# Autodesk Inventor assembly: søjle+vange
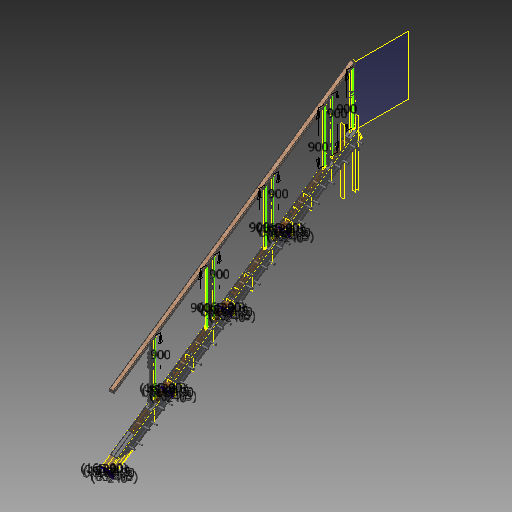
[picture p0: Inventor's stored thumbnail of the model, 512x512]
Saved by Autodesk Inventor 2018 (Build 220112000, 112)
## iProperties
Created: 2019-09-25
Part Number: søjle+vange
Document SubType Name: Assembly
Designer: Kristoffer Ek
Mass: 165952 g
Surface Area: 103178 cm^2
Volume: 42097.6 cm^3
Density: 3.94208 g/cm^3
Description: Beplantet bæredygtig trappe
Engineer: Kristoffer Ek
Authority: Loppen
Author: Kristoffer Ek
Title: Beplantet bæredygtig trappe
## Documents named in this file (35)
- Z:\trappe\søjle+vange.iam
- Z:\trappe\modul top.iam
- Z:\trappe\søjle\stilladssøjle.iam
- Z:\trappe\modul.iam
- Z:\trappe\modul bund.iam
- Z:\trappe\håndfang\træhåndfang.ipt
- Z:\trappe\hegn\hegnspæl.iam
- Z:\trappe\hegn\hegnspæl omvendt.iam
- Z:\trappe\søjle+vange\Design Accelerator\Bolted Connection1.iam
- Z:\trappe\søjle+vange\Design Accelerator\Bolted Connection2.iam
- Z:\trappe\søjle+vange\Design Accelerator\Bolted Connection3.iam
- Z:\trappe\søjle+vange\Design Accelerator\Bolted Connection4.iam
- Z:\trappe\søjle+vange\Design Accelerator\Bolted Connection5.iam
- Z:\trappe\søjle+vange\Design Accelerator\Bolted Connection6.iam
- Z:\trappe\søjle+vange\Design Accelerator\Bolted Connection7.iam
- Z:\trappe\søjle+vange\Design Accelerator\Bolted Connection8.iam
- Z:\trappe\søjle+vange\Design Accelerator\Bolted Connection9.iam
- Z:\trappe\søjle+vange\Design Accelerator\Bolted Connection10.iam
- Z:\trappe\søjle+vange\Design Accelerator\Bolted Connection11.iam
- Z:\trappe\søjle+vange\Design Accelerator\Bolted Connection12.iam
- Z:\trappe\søjle+vange\Design Accelerator\Bolted Connection13.iam
- Z:\trappe\søjle+vange\Design Accelerator\Bolted Connection14.iam
- Z:\trappe\søjle+vange\Design Accelerator\Bolted Connection15.iam
- Z:\trappe\søjle+vange\Design Accelerator\Bolted Connection16.iam
- Z:\trappe\søjle+vange\Design Accelerator\Bolted Connection17.iam
- Z:\trappe\søjle+vange\Design Accelerator\Bolted Connection18.iam
- Z:\trappe\søjle+vange\Design Accelerator\Bolted Connection19.iam
- Z:\trappe\søjle+vange\Design Accelerator\Bolted Connection20.iam
- Z:\trappe\søjle+vange\Design Accelerator\Bolted Connection21.iam
- Z:\trappe\søjle+vange\Design Accelerator\Bolted Connection22.iam
- Z:\trappe\søjle+vange\Design Accelerator\Bolted Connection23.iam
- Z:\trappe\søjle+vange\Design Accelerator\Bolted Connection24.iam
- Z:\trappe\hegn\hegnspæl, oppe, top.iam
- hegnspæl.iam
- Z:\trappe\håndfang\led-liste.ipt
## Components (39 placed, 9 different names)
1. stilladssøjle:2 [sub-assembly] — Mate:3, Mate:4, øre, Mate:14, Tangent:4
2. modul top:1 [sub-assembly] — Mate:3, Mate:4, øre, Flush:1, Flush:3, Mate:6, Mate:10, Mate:11, Flush:10, Tangent:1, Mate:13, Mate:24, Mate:26, Mate:28, Mate:30, Mate:32, Mate:34, Mate:36, Mate:38, Tangent:11, Mate:73, Mate:76, Mate:77
3. modul:1 [sub-assembly] — Flush:1, Flush:2, Flush:3, Flush:4, Mate:6, Mate:7, Flush:13, Mate:15, Tangent:5, Mate:23, Mate:25, Mate:27, Mate:29, Mate:31, Mate:33, Mate:35, Mate:37, Mate:48, Mate:50, Mate:52, Mate:54, Mate:74, Tangent:12, Mate:75
4. modul:2 [sub-assembly] — Flush:2, Flush:4, Mate:7, Flush:5, Flush:6, Flush:7, Mate:8, Flush:15, Mate:16, Mate:17, Tangent:7, Mate:39, Mate:40, Mate:41, Mate:42, Mate:43, Mate:44, Mate:45, Mate:46, Mate:47, Mate:49, Mate:51, Mate:53, Mate:56, Mate:58, Mate:60, Mate:62, Mate:64, Mate:66, Mate:68, Mate:70, Tangent:9, Mate:71
5. modul bund:1 [sub-assembly] — Flush:5, Flush:6, Flush:7, Mate:8, Mate:18, Mate:55, Mate:57, Mate:59, Mate:61, Mate:63, Mate:65, Mate:67, Mate:69, Tangent:10, Mate:72
6. træhåndfang:1 — Mate:10, Mate:76, Mate:77, Mate:78, Mate:79, Mate:80
7. hegnspæl:1 [sub-assembly] — Mate:11, Flush:10, Tangent:1
8. hegnspæl omvendt:1 [sub-assembly] — Mate:74, Tangent:12, Mate:75
9. hegnspæl:2 [sub-assembly] — Flush:13, Mate:15, Tangent:5
10. hegnspæl omvendt:2 [sub-assembly] — Mate:16, Tangent:9, Mate:71
11. hegnspæl:3 [sub-assembly] — Flush:15, Mate:17, Tangent:7
12. hegnspæl omvendt:3 [sub-assembly] — Mate:18, Tangent:10, Mate:72
13. hegnspæl:4 [sub-assembly] — Mate:14, Tangent:4
14. hegnspæl omvendt:4 [sub-assembly] — Mate:13, Tangent:11, Mate:73
15. Bolted Connection:1 [sub-assembly] — Mate:27, Mate:28
16. Bolted Connection:2 [sub-assembly] — Mate:29, Mate:30
17. Bolted Connection:3 [sub-assembly] — Mate:23, Mate:24
18. Bolted Connection:4 [sub-assembly] — Mate:25, Mate:26
19. Bolted Connection:5 [sub-assembly] — Mate:31, Mate:32
20. Bolted Connection:6 [sub-assembly] — Mate:33, Mate:34
21. Bolted Connection:7 [sub-assembly] — Mate:35, Mate:36
22. Bolted Connection:8 [sub-assembly] — Mate:37, Mate:38
23. Bolted Connection:9 [sub-assembly] — Mate:39, Mate:40
24. Bolted Connection:10 [sub-assembly] — Mate:41, Mate:42
25. Bolted Connection:11 [sub-assembly] — Mate:43, Mate:44
26. Bolted Connection:12 [sub-assembly] — Mate:45, Mate:46
27. Bolted Connection:13 [sub-assembly] — Mate:47, Mate:48
28. Bolted Connection:14 [sub-assembly] — Mate:49, Mate:50
29. Bolted Connection:15 [sub-assembly] — Mate:51, Mate:52
30. Bolted Connection:16 [sub-assembly] — Mate:53, Mate:54
31. Bolted Connection:17 [sub-assembly] — Mate:55, Mate:56
32. Bolted Connection:18 [sub-assembly] — Mate:57, Mate:58
33. Bolted Connection:19 [sub-assembly] — Mate:59, Mate:60
34. Bolted Connection:20 [sub-assembly] — Mate:61, Mate:62
35. Bolted Connection:21 [sub-assembly] — Mate:63, Mate:64
36. Bolted Connection:22 [sub-assembly] — Mate:65, Mate:66
37. Bolted Connection:23 [sub-assembly] — Mate:67, Mate:68
38. Bolted Connection:24 [sub-assembly] — Mate:69, Mate:70
39. led-liste:1 — Mate:78, Mate:79, Mate:80
## Relationships (91: Mate 73, Flush 10, Tangent 8)
- [Mate]: stilladssøjle:2 ↔ modul top:1
- Mate:3: stilladssøjle:2 ↔ modul top:1
- Mate:4: stilladssøjle:2 ↔ modul top:1
- øre [Mate]: stilladssøjle:2 ↔ modul top:1
- Flush:1: modul top:1 ↔ modul:1
- Flush:2: modul:1 ↔ modul:2
- Flush:3: modul top:1 ↔ modul:1
- Flush:4: modul:1 ↔ modul:2
- Mate:6 (2 mm): modul top:1 ↔ modul:1
- Mate:7 (2 mm): modul:1 ↔ modul:2
- Flush:5: modul:2 ↔ modul bund:1
- Flush:6: modul:2 ↔ modul bund:1
- Flush:7: modul:2 ↔ modul bund:1
- Mate:8 (2 mm): modul:2 ↔ modul bund:1
- Mate:10: modul top:1 ↔ træhåndfang:1
- Mate:11: modul top:1 ↔ hegnspæl:1
- Flush:10: modul top:1 ↔ hegnspæl:1
- Tangent:1: modul top:1 ↔ hegnspæl:1
- Mate:13: modul top:1 ↔ hegnspæl omvendt:4
- Mate:14: stilladssøjle:2 ↔ hegnspæl:4
- Tangent:4: stilladssøjle:2 ↔ hegnspæl:4
- Flush:13: modul:1 ↔ hegnspæl:2
- Flush:15: modul:2 ↔ hegnspæl:3
- Mate:15: modul:1 ↔ hegnspæl:2
- Tangent:5: modul:1 ↔ hegnspæl:2
- Mate:16: modul:2 ↔ hegnspæl omvendt:2
- Mate:17: modul:2 ↔ hegnspæl:3
- Mate:18: modul bund:1 ↔ hegnspæl omvendt:3
- Tangent:7: modul:2 ↔ hegnspæl:3
- Mate:23: modul:1 ↔ Bolted Connection:3
- Mate:24: modul top:1 ↔ Bolted Connection:3
- Mate:25: modul:1 ↔ Bolted Connection:4
- Mate:26: modul top:1 ↔ Bolted Connection:4
- Mate:27: modul:1 ↔ Bolted Connection:1
- Mate:28: modul top:1 ↔ Bolted Connection:1
- Mate:29: modul:1 ↔ Bolted Connection:2
- Mate:30: modul top:1 ↔ Bolted Connection:2
- Mate:31: modul:1 ↔ Bolted Connection:5
- Mate:32: modul top:1 ↔ Bolted Connection:5
- Mate:33: modul:1 ↔ Bolted Connection:6
- Mate:34: modul top:1 ↔ Bolted Connection:6
- Mate:35: modul:1 ↔ Bolted Connection:7
- Mate:36: modul top:1 ↔ Bolted Connection:7
- Mate:37: modul:1 ↔ Bolted Connection:8
- Mate:38: modul top:1 ↔ Bolted Connection:8
- Mate:39: modul:2 ↔ Bolted Connection:9
- Mate:40: modul:2 ↔ Bolted Connection:9
- Mate:41: modul:2 ↔ Bolted Connection:10
- Mate:42: modul:2 ↔ Bolted Connection:10
- Mate:43: modul:2 ↔ Bolted Connection:11
- Mate:44: modul:2 ↔ Bolted Connection:11
- Mate:45: modul:2 ↔ Bolted Connection:12
- Mate:46: modul:2 ↔ Bolted Connection:12
- Mate:47: modul:2 ↔ Bolted Connection:13
- Mate:48: modul:1 ↔ Bolted Connection:13
- Mate:49: modul:2 ↔ Bolted Connection:14
- Mate:50: modul:1 ↔ Bolted Connection:14
- Mate:51: modul:2 ↔ Bolted Connection:15
- Mate:52: modul:1 ↔ Bolted Connection:15
- Mate:53: modul:2 ↔ Bolted Connection:16
- Mate:54: modul:1 ↔ Bolted Connection:16
- Mate:55: modul bund:1 ↔ Bolted Connection:17
- Mate:56: modul:2 ↔ Bolted Connection:17
- Mate:57: modul bund:1 ↔ Bolted Connection:18
- Mate:58: modul:2 ↔ Bolted Connection:18
- Mate:59: modul bund:1 ↔ Bolted Connection:19
- Mate:60: modul:2 ↔ Bolted Connection:19
- Mate:61: modul bund:1 ↔ Bolted Connection:20
- Mate:62: modul:2 ↔ Bolted Connection:20
- Mate:63: modul bund:1 ↔ Bolted Connection:21
- Mate:64: modul:2 ↔ Bolted Connection:21
- Mate:65: modul bund:1 ↔ Bolted Connection:22
- Mate:66: modul:2 ↔ Bolted Connection:22
- Mate:67: modul bund:1 ↔ Bolted Connection:23
- Mate:68: modul:2 ↔ Bolted Connection:23
- Mate:69: modul bund:1 ↔ Bolted Connection:24
- Mate:70: modul:2 ↔ Bolted Connection:24
- Tangent:9: modul:2 ↔ hegnspæl omvendt:2
- Mate:71: modul:2 ↔ hegnspæl omvendt:2
- Tangent:10: modul bund:1 ↔ hegnspæl omvendt:3
- Mate:72: modul bund:1 ↔ hegnspæl omvendt:3
- Tangent:11: modul top:1 ↔ hegnspæl omvendt:4
- Mate:73: modul top:1 ↔ hegnspæl omvendt:4
- Mate:74: modul:1 ↔ hegnspæl omvendt:1
- Tangent:12: modul:1 ↔ hegnspæl omvendt:1
- Mate:75: modul:1 ↔ hegnspæl omvendt:1
- Mate:76: modul top:1 ↔ træhåndfang:1
- Mate:77 (1.5 mm): modul top:1 ↔ træhåndfang:1
- Mate:78: træhåndfang:1 ↔ led-liste:1
- Mate:79: træhåndfang:1 ↔ led-liste:1
- Mate:80: træhåndfang:1 ↔ led-liste:1
